# Autodesk Inventor assembly: Robot
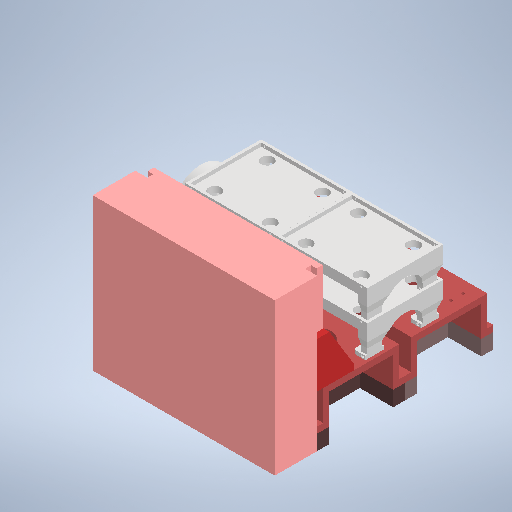
[picture p0: Inventor's stored thumbnail of the model, 512x512]
Saved by Autodesk Inventor 2025.3 (Build 293356000, 356)
## iProperties
Created: 2025-04-27
Part Number: Robot
Document SubType Name: Assembly
Designer: SEON
Author: SEON
## Documents named in this file (8)
- C:\Users\SEON\Documents\Inventor\LastCapstone\Robot.iam
- C:\Users\SEON\Documents\Inventor\LastCapstone\DummyModule.ipt
- C:\Users\SEON\Documents\Inventor\LastCapstone\RobotBase.ipt
- C:\Users\SEON\Documents\Inventor\LastCapstone\ModuleConnector.ipt
- C:\Users\SEON\Documents\Inventor\LastCapstone\DummyWheel.ipt
- C:\Users\SEON\Documents\Inventor\LastCapstone\WheelCorver.ipt
- C:\Users\SEON\Documents\Inventor\LastCapstone\partContainer.ipt
- C:\Users\SEON\Documents\Inventor\LastCapstone\partContainerConnector.ipt
## Components (23 placed, 7 different names)
1. RobotBase:1 — 메이트:1, 메이트:4, 메이트:5, 메이트:6, 플러쉬:3, 메이트:9, 플러쉬:4, 메이트:11, 메이트:12, 플러쉬:5, 플러쉬:6, 메이트:13, 플러쉬:8, 플러쉬:17, 메이트:29, 플러쉬:18
2. DummyModule:1 — 메이트:6, 메이트:8, 메이트:18, 메이트:19
3. ModuleConnector:1 — 플러쉬:3, 메이트:8, 메이트:10, 메이트:16, 메이트:18, 메이트:19
4. DummyWheel:1 — 각도:1
5. WheelCorver:1 — 메이트:9, 메이트:10, 플러쉬:4, 메이트:16, 플러쉬:10, 플러쉬:11, 메이트:17, 메이트:21, 플러쉬:14, 메이트:30, 메이트:34, 메이트:41
6. WheelCorver:2 — 메이트:11, 플러쉬:11, 메이트:17, 메이트:26, 메이트:33, 메이트:37, 메이트:38
7. RobotBase:2 — 메이트:13, 메이트:15, 플러쉬:7, 플러쉬:8, 플러쉬:10
8. RobotBase:3 — 메이트:14, 메이트:15, 플러쉬:7, 플러쉬:9
9. RobotBase:4 — 메이트:12, 플러쉬:5, 플러쉬:6, 메이트:14, 플러쉬:9, 메이트:28, 플러쉬:15, 플러쉬:16
10. partContainer:1 — 메이트:20, 플러쉬:12, 플러쉬:13, 메이트:21, 플러쉬:14, 메이트:25, 메이트:27, 메이트:31, 메이트:32, 메이트:35, 메이트:36, 메이트:39, 메이트:40, 메이트:42, 메이트:44, 메이트:45
11. partContainer:2 — 메이트:20, 플러쉬:12, 플러쉬:13, 메이트:43, 메이트:46, 메이트:47, 메이트:48, 메이트:49, 메이트:51, 메이트:52, 메이트:54, 메이트:55, 플러쉬:19, 메이트:56, 플러쉬:20, 메이트:57
12. partContainer:4 — 메이트:43, 메이트:46, 메이트:47
13. partContainerConnector:1 — 메이트:25, 메이트:26, 메이트:27, 메이트:33
14. WheelCorver:3 — 메이트:28, 플러쉬:15, 플러쉬:16, 메이트:50
15. WheelCorver:4 — 플러쉬:17, 메이트:29, 플러쉬:18, 메이트:53
16. partContainerConnector:2 — 메이트:30, 메이트:31, 메이트:32, 메이트:34
17. partContainerConnector:3 — 메이트:35, 메이트:36, 메이트:37, 메이트:38
18. partContainerConnector:4 — 메이트:39, 메이트:40, 메이트:41
19. partContainer:5 — 메이트:42, 메이트:44, 메이트:45
20. partContainerConnector:5 — 메이트:48, 메이트:49, 메이트:50
21. partContainerConnector:6 — 메이트:51, 메이트:52, 메이트:53
22. partContainerConnector:7 — 메이트:56, 플러쉬:20, 메이트:57
23. partContainerConnector:8 — 메이트:54, 메이트:55, 플러쉬:19
## Relationships (70: Mate 51, Flush 18, Angle 1)
- 메이트:1 [Mate]: RobotBase:1
- 메이트:4 [Mate]: RobotBase:1
- 메이트:5 [Mate]: RobotBase:1
- 메이트:6 [Mate]: RobotBase:1 ↔ DummyModule:1
- 플러쉬:3 [Flush]: RobotBase:1 ↔ ModuleConnector:1
- 메이트:8 [Mate]: DummyModule:1 ↔ ModuleConnector:1
- 각도:1 [Angle] (0 deg): DummyWheel:1
- 메이트:9 [Mate]: RobotBase:1 ↔ WheelCorver:1
- 메이트:10 [Mate]: ModuleConnector:1 ↔ WheelCorver:1
- 플러쉬:4 [Flush]: RobotBase:1 ↔ WheelCorver:1
- 메이트:11 [Mate]: RobotBase:1 ↔ WheelCorver:2
- 메이트:12 [Mate]: RobotBase:1 ↔ RobotBase:4
- 플러쉬:5 [Flush]: RobotBase:1 ↔ RobotBase:4
- 플러쉬:6 [Flush]: RobotBase:1 ↔ RobotBase:4
- 메이트:13 [Mate]: RobotBase:1 ↔ RobotBase:2
- 메이트:14 [Mate]: RobotBase:3 ↔ RobotBase:4
- 메이트:15 [Mate]: RobotBase:2 ↔ RobotBase:3
- 플러쉬:7 [Flush]: RobotBase:2 ↔ RobotBase:3
- 플러쉬:8 [Flush]: RobotBase:1 ↔ RobotBase:2
- 플러쉬:9 [Flush]: RobotBase:3 ↔ RobotBase:4
- 메이트:16 [Mate]: ModuleConnector:1 ↔ WheelCorver:1
- 플러쉬:10 [Flush]: WheelCorver:1 ↔ RobotBase:2
- 플러쉬:11 [Flush]: WheelCorver:1 ↔ WheelCorver:2
- 메이트:17 [Mate]: WheelCorver:1 ↔ WheelCorver:2
- 메이트:18 [Mate]: DummyModule:1 ↔ ModuleConnector:1
- 메이트:19 [Mate]: DummyModule:1 ↔ ModuleConnector:1
- 메이트:20 [Mate]: partContainer:1 ↔ partContainer:2
- 플러쉬:12 [Flush]: partContainer:1 ↔ partContainer:2
- 플러쉬:13 [Flush]: partContainer:1 ↔ partContainer:2
- 메이트:21 [Mate]: WheelCorver:1 ↔ partContainer:1
- 플러쉬:14 [Flush]: WheelCorver:1 ↔ partContainer:1
- 메이트:25 [Mate]: partContainer:1 ↔ partContainerConnector:1
- 메이트:26 [Mate]: WheelCorver:2 ↔ partContainerConnector:1
- 메이트:27 [Mate]: partContainer:1 ↔ partContainerConnector:1
- 메이트:28 [Mate]: RobotBase:4 ↔ WheelCorver:3
- 플러쉬:15 [Flush]: RobotBase:4 ↔ WheelCorver:3
- 플러쉬:16 [Flush]: RobotBase:4 ↔ WheelCorver:3
- 플러쉬:17 [Flush]: RobotBase:1 ↔ WheelCorver:4
- 메이트:29 [Mate]: RobotBase:1 ↔ WheelCorver:4
- 플러쉬:18 [Flush]: RobotBase:1 ↔ WheelCorver:4
- 메이트:30 [Mate]: WheelCorver:1 ↔ partContainerConnector:2
- 메이트:31 [Mate]: partContainer:1 ↔ partContainerConnector:2
- 메이트:32 [Mate]: partContainer:1 ↔ partContainerConnector:2
- 메이트:33 [Mate]: WheelCorver:2 ↔ partContainerConnector:1
- 메이트:34 [Mate]: WheelCorver:1 ↔ partContainerConnector:2
- 메이트:35 [Mate]: partContainer:1 ↔ partContainerConnector:3
- 메이트:36 [Mate]: partContainer:1 ↔ partContainerConnector:3
- 메이트:37 [Mate]: WheelCorver:2 ↔ partContainerConnector:3
- 메이트:38 [Mate]: WheelCorver:2 ↔ partContainerConnector:3
- 메이트:39 [Mate]: partContainer:1 ↔ partContainerConnector:4
- 메이트:40 [Mate]: partContainer:1 ↔ partContainerConnector:4
- 메이트:41 [Mate]: WheelCorver:1 ↔ partContainerConnector:4
- 메이트:42 [Mate]: partContainer:1 ↔ partContainer:5
- 메이트:43 [Mate]: partContainer:2 ↔ partContainer:4
- 메이트:44 [Mate] (0.5 mm): partContainer:1 ↔ partContainer:5
- 메이트:45 [Mate] (0.5 mm): partContainer:1 ↔ partContainer:5
- 메이트:46 [Mate] (0.5 mm): partContainer:2 ↔ partContainer:4
- 메이트:47 [Mate] (0.5 mm): partContainer:2 ↔ partContainer:4
- 메이트:48 [Mate]: partContainer:2 ↔ partContainerConnector:5
- 메이트:49 [Mate]: partContainer:2 ↔ partContainerConnector:5
- 메이트:50 [Mate]: WheelCorver:3 ↔ partContainerConnector:5
- 메이트:51 [Mate]: partContainer:2 ↔ partContainerConnector:6
- 메이트:52 [Mate]: partContainer:2 ↔ partContainerConnector:6
- 메이트:53 [Mate]: WheelCorver:4 ↔ partContainerConnector:6
- 메이트:54 [Mate]: partContainer:2 ↔ partContainerConnector:8
- 메이트:55 [Mate]: partContainer:2 ↔ partContainerConnector:8
- 플러쉬:19 [Flush]: partContainer:2 ↔ partContainerConnector:8
- 메이트:56 [Mate]: partContainer:2 ↔ partContainerConnector:7
- 플러쉬:20 [Flush]: partContainer:2 ↔ partContainerConnector:7
- 메이트:57 [Mate]: partContainer:2 ↔ partContainerConnector:7
